# Autodesk Inventor assembly: shoulder
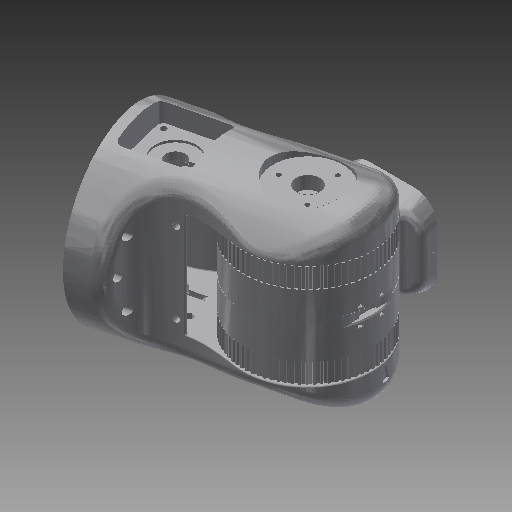
[picture p0: Inventor's stored thumbnail of the model, 512x512]
Saved by Autodesk Inventor 2019 (Build 230136000, 136)
## iProperties
Created: 2020-03-22
Part Number: shoulder
Document SubType Name: Assembly
Designer: james
Author: james
## Documents named in this file (4)
- F:\JimsRobot\FIRSTRobots\Design\RBX1-REMIX\shoulder\shoulder.iam
- F:\JimsRobot\FIRSTRobots\Design\RBX1-REMIX\shoulder\shoulder_gear_left_qty1.ipt
- F:\JimsRobot\FIRSTRobots\Design\RBX1-REMIX\shoulder\shoulder_gear_right_qty1.ipt
- F:\JimsRobot\FIRSTRobots\Design\RBX1-REMIX\shoulder\shoulder_qty1.ipt
## Components (3 placed, 3 different names)
1. shoulder_gear_left_qty1:1 — Mate:1, Flush:1, Flush:2, Mate:2, Mate:3
2. shoulder_gear_right_qty1:1 — Mate:1, Flush:1, Flush:2
3. shoulder_qty1:1 — Mate:2, Mate:3
## Relationships (5: Mate 3, Flush 2)
- Mate:1: shoulder_gear_left_qty1:1 ↔ shoulder_gear_right_qty1:1
- Flush:1: shoulder_gear_left_qty1:1 ↔ shoulder_gear_right_qty1:1
- Flush:2: shoulder_gear_left_qty1:1 ↔ shoulder_gear_right_qty1:1
- Mate:2: shoulder_gear_left_qty1:1 ↔ shoulder_qty1:1
- Mate:3: shoulder_gear_left_qty1:1 ↔ shoulder_qty1:1
